# Autodesk Inventor assembly: climber
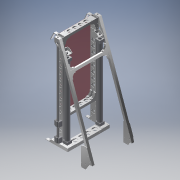
[picture p0: Inventor's stored thumbnail of the model, 180x180]
Saved by Autodesk Inventor 2019.4 (Build 234330000, 330)
## iProperties
Created: 2020-01-07
Part Number: climber
Document SubType Name: Assembly
Designer: Mark
Mass: 13923.9 g
Surface Area: 29345.8 cm^2
Volume: 6495.57 cm^3
Density: 2.1436 g/cm^3
Author: Mark
## Documents named in this file (19)
- C:\Users\admin\Desktop\FRC 2020 Engineering\GitHub\7738-2020\Elevator Mechanism\climber.iam
- C:\Users\admin\Desktop\FRC 2020 Engineering\GitHub\7738-2020\Elevator Mechanism\Extrusion Mid.ipt
- C:\Users\admin\Desktop\FRC 2020 Engineering\GitHub\7738-2020\Elevator Mechanism\climber\Design Accelerator\Shaft2.iam
- C:\Users\admin\Desktop\FRC 2020 Engineering\GitHub\7738-2020\Elevator Mechanism\Base.ipt
- C:\Users\admin\Desktop\FRC 2020 Engineering\GitHub\7738-2020\Elevator Mechanism\Standard Bracing.ipt
- C:\Users\admin\Desktop\FRC 2020 Engineering\GitHub\7738-2020\Elevator Mechanism\Top Connector.ipt
- C:\Users\admin\Desktop\FRC 2020 Engineering\GitHub\7738-2020\Elevator Mechanism\Elevator Support.ipt
- C:\Users\admin\Desktop\FRC 2020 Engineering\GitHub\7738-2020\Elevator Mechanism\Top Support.ipt
- C:\Users\admin\Desktop\FRC 2020 Engineering\GitHub\7738-2020\Elevator Mechanism\Lifting Part.iam
- C:\Users\admin\Desktop\FRC 2020 Engineering\GitHub\7738-2020\Elevator Mechanism\Линейный подшипник SCS 20UU.ipt
- C:\Users\admin\Desktop\FRC 2020 Engineering\GitHub\7738-2020\Elevator Mechanism\SC40 700 Assembly.iam
- C:\Users\admin\Desktop\FRC 2020 Engineering\GitHub\7738-2020\Elevator Mechanism\Steel Bracing.ipt
- C:\Users\admin\Desktop\FRC 2020 Engineering\GitHub\7738-2020\Elevator Mechanism\Pneumatic Upper Support.ipt
- C:\Users\admin\Desktop\FRC 2020 Engineering\GitHub\7738-2020\Elevator Mechanism\Sheet Metal Support Thing.ipt
- C:\Users\admin\Desktop\FRC 2020 Engineering\GitHub\7738-2020\Elevator Mechanism\Custom Bracket.ipt
- C:\Users\admin\Desktop\FRC 2020 Engineering\GitHub\7738-2020\Elevator Mechanism\climber\AIP\FEA\d484goxmo.fins
- C:\Users\admin\Desktop\FRC 2020 Engineering\GitHub\7738-2020\Elevator Mechanism\climber\AIP\FEA\d484goxmo.fsat
- C:\Users\admin\Desktop\FRC 2020 Engineering\GitHub\7738-2020\Elevator Mechanism\climber\AIP\FEA\d484goxmo.ftes
- C:\Users\admin\Desktop\FRC 2020 Engineering\GitHub\7738-2020\Elevator Mechanism\climber\AIP\FEA\d484goxmo.fwiz
## Components (31 placed, 14 different names)
1. Extrusion Mid:1 — Mate:10, Flush:3, Flush:4, Mate:76, Flush:18, Mate:77, Flush:20, Mate:90, Mate:92, Mate:93
2. Shaft:1 [sub-assembly] — Mate:7, Mate:20, Mate:21, Mate:39, Mate:40, Flush:31
3. Shaft:2 [sub-assembly] — Mate:6, Flush:1, Mate:26, Mate:27, Cylindrical:1, Mate:52
4. Base:1 — Mate:6, Flush:1, Mate:9, Flush:2, Mate:10, Flush:3, Flush:4, Flush:5, Flush:16, Mate:64, Flush:21, Mate:78, Mate:79, Mate:80, Mate:89, Flush:32
5. Base:2 — Mate:7, Mate:9, Flush:2, Flush:5, Mate:51, Mate:74, Flush:19, Mate:81, Mate:82, Flush:22, Flush:31, Mate:91
6. Standard Bracing:1 — Mate:74
7. Standard Bracing:4 — Mate:64
8. Top Connector:1 — Mate:20, Mate:21, Flush:8, Mate:59, Mate:60
9. Elevator Support:1 — Flush:8, Mate:28, Flush:11, Mate:36, Mate:37, Mate:59, Mate:60, Mate:85, Mate:86, Mate:87
10. Top Connector:2 — Mate:26, Mate:27, Mate:57, Mate:58
11. Elevator Support:2 — Mate:57, Flush:16, Mate:58, Mate:62, Mate:63, Flush:17, Mate:88
12. Top Support:1 — Mate:28, Flush:11, Mate:31, Mate:32, Mate:33, Mate:38, Mate:61
13. Standard Bracing:5 — Mate:32, Mate:33, Mate:62
14. Standard Bracing:6 — Mate:31, Mate:63, Flush:17
15. Standard Bracing:7 — Flush:12, Mate:35, Flush:13
16. Standard Bracing:8 — Flush:12, Mate:35, Flush:13, Mate:36, Mate:37, Mate:38, Mate:61
17. Lifting Part:1 [sub-assembly] — Mate:53, Mate:54, Flush:15, Mate:55, Mate:56, Flush:23, Flush:24
18. Линейный подшипник SCS 20UU:1 — Mate:39, Mate:56
19. Линейный подшипник SCS 20UU:2 — Mate:40, Mate:55
20. Линейный подшипник SCS 20UU:3 — Mate:43, Flush:14, Cylindrical:1
21. Линейный подшипник SCS 20UU:4 — Mate:43, Flush:14, Mate:52, Mate:53, Mate:54, Flush:15
22. SC40 700 Assembly:1 [sub-assembly] — Mate:76, Flush:18, Flush:19, Flush:23, Mate:83, Flush:25, Flush:26
23. SC40 700 Assembly:2 [sub-assembly] — Mate:77, Flush:20, Flush:21, Flush:24, Mate:84, Flush:27, Flush:28
24. Steel Bracing:1 — Mate:78, Mate:79, Mate:80
25. Steel Bracing:2 — Mate:81, Mate:82, Flush:22
26. Pneumatic Upper Support:1 — Mate:83, Flush:25, Flush:26
27. Pneumatic Upper Support:2 — Mate:84, Flush:27, Flush:28
28. Sheet Metal Support Thing:1 — Mate:85, Mate:86, Mate:87, Flush:29, Flush:30
29. Sheet Metal Support Thing:2 — Mate:88, Flush:29, Flush:30
30. Custom Bracket:1 — Mate:89, Mate:90, Flush:32
31. Custom Bracket:2 — Mate:91, Mate:92, Mate:93
## Relationships (81: Mate 52, Flush 28, CylindricalJoint 1)
- Mate:6: Shaft:2 ↔ Base:1
- Flush:1: Shaft:2 ↔ Base:1
- Mate:7: Shaft:1 ↔ Base:2
- Mate:9 (400 mm): Base:1 ↔ Base:2
- Flush:2: Base:1 ↔ Base:2
- Mate:10: Extrusion Mid:1 ↔ Base:1
- Flush:3: Extrusion Mid:1 ↔ Base:1
- Flush:4 (155 mm): Extrusion Mid:1 ↔ Base:1
- Flush:5: Base:1 ↔ Base:2
- Mate:20: Shaft:1 ↔ Top Connector:1
- Mate:21: Shaft:1 ↔ Top Connector:1
- Flush:8: Top Connector:1 ↔ Elevator Support:1
- Mate:26: Shaft:2 ↔ Top Connector:2
- Mate:27: Shaft:2 ↔ Top Connector:2
- Mate:28: Elevator Support:1 ↔ Top Support:1
- Flush:11: Elevator Support:1 ↔ Top Support:1
- Mate:31: Top Support:1 ↔ Standard Bracing:6
- Mate:32: Top Support:1 ↔ Standard Bracing:5
- Mate:33: Top Support:1 ↔ Standard Bracing:5
- Flush:12: Standard Bracing:7 ↔ Standard Bracing:8
- Mate:35 (25 mm): Standard Bracing:7 ↔ Standard Bracing:8
- Flush:13: Standard Bracing:7 ↔ Standard Bracing:8
- Mate:36: Elevator Support:1 ↔ Standard Bracing:8
- Mate:37: Elevator Support:1 ↔ Standard Bracing:8
- Mate:38: Top Support:1 ↔ Standard Bracing:8
- Mate:39: Shaft:1 ↔ Линейный подшипник SCS 20UU:1
- Mate:40: Shaft:1 ↔ Линейный подшипник SCS 20UU:2
- Mate:43 (100 mm): Линейный подшипник SCS 20UU:3 ↔ Линейный подшипник SCS 20UU:4
- Flush:14: Линейный подшипник SCS 20UU:3 ↔ Линейный подшипник SCS 20UU:4
- Cylindrical:1: Shaft:2 ↔ Линейный подшипник SCS 20UU:3
- Mate:51: Base:2
- Mate:52: Shaft:2 ↔ Линейный подшипник SCS 20UU:4
- Mate:53: Lifting Part:1 ↔ Линейный подшипник SCS 20UU:4
- Mate:54: Lifting Part:1 ↔ Линейный подшипник SCS 20UU:4
- Flush:15: Lifting Part:1 ↔ Линейный подшипник SCS 20UU:4
- Mate:55: Lifting Part:1 ↔ Линейный подшипник SCS 20UU:2
- Mate:56: Lifting Part:1 ↔ Линейный подшипник SCS 20UU:1
- Mate:57: Top Connector:2 ↔ Elevator Support:2
- Flush:16: Base:1 ↔ Elevator Support:2
- Mate:58: Top Connector:2 ↔ Elevator Support:2
- Mate:59: Top Connector:1 ↔ Elevator Support:1
- Mate:60: Top Connector:1 ↔ Elevator Support:1
- Mate:61: Top Support:1 ↔ Standard Bracing:8
- Mate:62: Elevator Support:2 ↔ Standard Bracing:5
- Mate:63: Elevator Support:2 ↔ Standard Bracing:6
- Flush:17: Elevator Support:2 ↔ Standard Bracing:6
- Mate:64: Base:1 ↔ Standard Bracing:4
- Mate:74: Base:2 ↔ Standard Bracing:1
- Mate:76 (3 mm): Extrusion Mid:1 ↔ SC40 700 Assembly:1
- Flush:18: Extrusion Mid:1 ↔ SC40 700 Assembly:1
- Flush:19 (25 mm): Base:2 ↔ SC40 700 Assembly:1
- Mate:77 (3 mm): Extrusion Mid:1 ↔ SC40 700 Assembly:2
- Flush:20: Extrusion Mid:1 ↔ SC40 700 Assembly:2
- Flush:21 (25 mm): Base:1 ↔ SC40 700 Assembly:2
- Mate:78: Base:1 ↔ Steel Bracing:1
- Mate:79: Base:1 ↔ Steel Bracing:1
- Mate:80: Base:1 ↔ Steel Bracing:1
- Mate:81: Base:2 ↔ Steel Bracing:2
- Mate:82: Base:2 ↔ Steel Bracing:2
- Flush:22: Base:2 ↔ Steel Bracing:2
- Flush:23 (-11.8 mm): Lifting Part:1 ↔ SC40 700 Assembly:1
- Flush:24 (-11.8 mm): Lifting Part:1 ↔ SC40 700 Assembly:2
- Mate:83: SC40 700 Assembly:1 ↔ Pneumatic Upper Support:1
- Flush:25: SC40 700 Assembly:1 ↔ Pneumatic Upper Support:1
- Flush:26: SC40 700 Assembly:1 ↔ Pneumatic Upper Support:1
- Mate:84: SC40 700 Assembly:2 ↔ Pneumatic Upper Support:2
- Flush:27: SC40 700 Assembly:2 ↔ Pneumatic Upper Support:2
- Flush:28: SC40 700 Assembly:2 ↔ Pneumatic Upper Support:2
- Mate:85: Elevator Support:1 ↔ Sheet Metal Support Thing:1
- Mate:86: Elevator Support:1 ↔ Sheet Metal Support Thing:1
- Mate:87: Elevator Support:1 ↔ Sheet Metal Support Thing:1
- Mate:88: Elevator Support:2 ↔ Sheet Metal Support Thing:2
- Flush:29: Sheet Metal Support Thing:1 ↔ Sheet Metal Support Thing:2
- Flush:30: Sheet Metal Support Thing:1 ↔ Sheet Metal Support Thing:2
- Flush:31: Shaft:1 ↔ Base:2
- Mate:89: Base:1 ↔ Custom Bracket:1
- Mate:90: Extrusion Mid:1 ↔ Custom Bracket:1
- Flush:32 (2.5 mm): Base:1 ↔ Custom Bracket:1
- Mate:91: Base:2 ↔ Custom Bracket:2
- Mate:92: Extrusion Mid:1 ↔ Custom Bracket:2
- Mate:93: Extrusion Mid:1 ↔ Custom Bracket:2
## Named parameters: sa_0 = 50000
note: some values were not read from the file. Shown as the stored number, unit unknown: "sa_0".
